# Autodesk Inventor assembly: FinalShooting
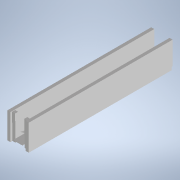
[picture p0: Inventor's stored thumbnail of the model, 180x180]
Saved by Autodesk Inventor 2020 (Build 240168000, 168)
## iProperties
Created: 2021-02-07
Part Number: FinalShooting
Document SubType Name: Assembly
Designer: moham
Author: moham
## Documents named in this file (7)
- D:\Projects\MCT 131\The project\shooting 3\FinalShooting.iam
- D:\Projects\MCT 131\The project\shooting 3\Base_1.ipt
- D:\Projects\MCT 131\The project\shooting 3\Side_2.ipt
- D:\Projects\MCT 131\The project\shooting 3\hOLD_2.ipt
- D:\Projects\MCT 131\The project\shooting 3\Sides_2.ipt
- D:\Projects\MCT 131\The project\shooting 3\Push_1.ipt
- D:\Projects\MCT 131\The project\shooting 3\Ruler_1.ipt
## Components (9 placed, 6 different names)
1. Base_1:1 — Mate:1, Flush:1, Flush:2, Mate:2, Flush:3, Flush:4, Flush:11, Flush:12, Flush:14, Mate:6, Mate:7, Mate:9, Flush:18, Mate:11, Flush:20
2. Side_2:1 — Mate:1, Flush:1, Flush:2, Flush:13, Mate:3
3. Side_2:2 — Mate:2, Flush:3, Flush:4, Mate:4, Flush:15, Flush:19
4. Sides_2:1 — Mate:4, Flush:14, Flush:15, Flush:17, Mate:8
5. Sides_2:2 — Flush:11, Flush:12, Flush:13, Mate:3, Mate:5, Flush:16
6. hOLD_2:1 — Flush:17, Mate:7, Mate:8
7. hOLD_2:2 — Mate:5, Mate:6, Flush:16, Mate:10
8. Push_1:1 — Mate:9, Flush:18, Flush:19
9. Ruler_1:1 — Mate:10, Mate:11, Flush:20
## Relationships (25: Flush 14, Mate 11)
- Mate:1: Base_1:1 ↔ Side_2:1
- Flush:1: Base_1:1 ↔ Side_2:1
- Flush:2: Base_1:1 ↔ Side_2:1
- Mate:2: Base_1:1 ↔ Side_2:2
- Flush:3: Base_1:1 ↔ Side_2:2
- Flush:4: Base_1:1 ↔ Side_2:2
- Flush:11: Base_1:1 ↔ Sides_2:2
- Flush:12: Base_1:1 ↔ Sides_2:2
- Flush:13: Side_2:1 ↔ Sides_2:2
- Mate:3: Side_2:1 ↔ Sides_2:2
- Mate:4: Side_2:2 ↔ Sides_2:1
- Flush:14: Base_1:1 ↔ Sides_2:1
- Flush:15: Side_2:2 ↔ Sides_2:1
- Mate:5: Sides_2:2 ↔ hOLD_2:2
- Mate:6: Base_1:1 ↔ hOLD_2:2
- Flush:16: Sides_2:2 ↔ hOLD_2:2
- Flush:17: Sides_2:1 ↔ hOLD_2:1
- Mate:7: Base_1:1 ↔ hOLD_2:1
- Mate:8: Sides_2:1 ↔ hOLD_2:1
- Mate:9 (2 mm): Base_1:1 ↔ Push_1:1
- Flush:18: Base_1:1 ↔ Push_1:1
- Flush:19: Side_2:2 ↔ Push_1:1
- Mate:10: hOLD_2:2 ↔ Ruler_1:1
- Mate:11: Base_1:1 ↔ Ruler_1:1
- Flush:20: Base_1:1 ↔ Ruler_1:1
